# Autodesk Inventor assembly: ASY GnG frame 2
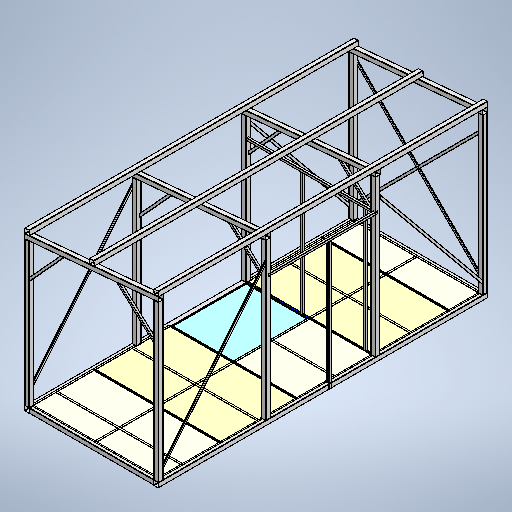
[picture p0: Inventor's stored thumbnail of the model, 512x512]
Saved by Autodesk Inventor 2025 (Build 290162010, 162A)
## iProperties
_SolveAssemblyDoc: Frame Generator Solve Assembly
_Version: 25.0.0
Created: 2025-10-19
Part Number: ASY GnG frame 2
Document SubType Name: Assembly
Designer: admin
Author: admin
## Documents named in this file (9)
- C:\Users\admin\Yandex.Disk\home pc\Inventor\GnG_Gantul_hill\ASY GnG frame 2.iam
- C:\Users\admin\Yandex.Disk\home pc\Inventor\GnG_Gantul_hill\GnG frame 2 sketch.ipt
- C:\Users\admin\Yandex.Disk\home pc\Inventor\GnG_Gantul_hill\ASY GnG frame 2\Frame\Frame 1760870485440.iam
- C:\Users\admin\Yandex.Disk\home pc\Inventor\GnG_Gantul_hill\GnG frame 2 floor sheet 5.ipt
- C:\Users\admin\Yandex.Disk\home pc\Inventor\GnG_Gantul_hill\GnG frame 2 floor sheet 6.ipt
- C:\Users\admin\Yandex.Disk\home pc\Inventor\GnG_Gantul_hill\GnG frame 2 floor sheet 7.ipt
- C:\Users\admin\Yandex.Disk\home pc\Inventor\GnG_Gantul_hill\GnG frame 2 floor sheet 8.ipt
- C:\Users\admin\Yandex.Disk\home pc\Inventor\GnG_Gantul_hill\GnG frame 2 floor sheet 9.ipt
- C:\Users\admin\Yandex.Disk\home pc\Inventor\GnG_Gantul_hill\GnG frame 2 floor sheet 10.ipt
## Components (8 placed, 8 different names)
1. GnG frame 2 sketch:1
2. Frame 1760870485440:1 [sub-assembly] — Mate:1, Mate:2, Mate:3, Flush:6, Mate:6, Mate:7
3. GnG frame 2 floor sheet 5:1 — Mate:1, Mate:2, Mate:3
4. GnG frame 2 floor sheet 6:1 — Flush:6, Rigid:1, Rigid:4, Mate:6
5. GnG frame 2 floor sheet 7:1 — Rigid:1, Rigid:2, Mate:7
6. GnG frame 2 floor sheet 8:1 — Rigid:2, Rigid:3
7. GnG frame 2 floor sheet 9:1 — Rigid:3
8. GnG frame 2 floor sheet 10:1 — Rigid:4
## Relationships (10: Mate 5, WeldJoint 4, Flush 1)
- Mate:1 (-20 mm): Frame 1760870485440:1 ↔ GnG frame 2 floor sheet 5:1
- Mate:2: Frame 1760870485440:1 ↔ GnG frame 2 floor sheet 5:1
- Mate:3: Frame 1760870485440:1 ↔ GnG frame 2 floor sheet 5:1
- Flush:6 (25 mm): Frame 1760870485440:1 ↔ GnG frame 2 floor sheet 6:1
- Rigid:1 [WeldJoint] (10 mm): GnG frame 2 floor sheet 6:1 ↔ GnG frame 2 floor sheet 7:1
- Rigid:2 [WeldJoint] (10 mm): GnG frame 2 floor sheet 7:1 ↔ GnG frame 2 floor sheet 8:1
- Rigid:3 [WeldJoint] (10 mm): GnG frame 2 floor sheet 8:1 ↔ GnG frame 2 floor sheet 9:1
- Rigid:4 [WeldJoint] (10 mm): GnG frame 2 floor sheet 6:1 ↔ GnG frame 2 floor sheet 10:1
- Mate:6: Frame 1760870485440:1 ↔ GnG frame 2 floor sheet 6:1
- Mate:7 (-30 mm): Frame 1760870485440:1 ↔ GnG frame 2 floor sheet 7:1
